# Autodesk Inventor assembly: boto suction pump
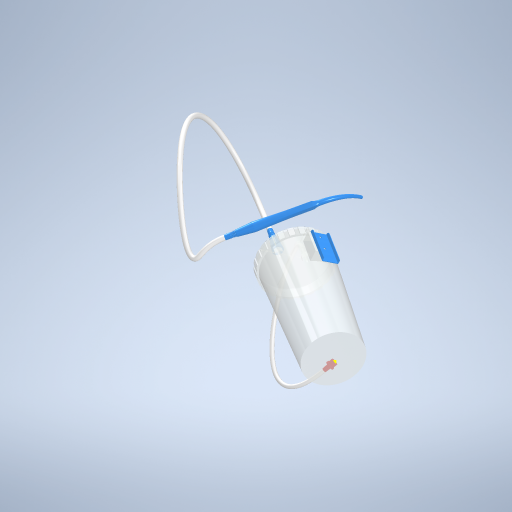
[picture p0: Inventor's stored thumbnail of the model, 512x512]
Saved by Autodesk Inventor 2024 (Build 280153000, 153)
## iProperties
Created: 2023-03-28
Part Number: boto suction pump
Description: STEP AP203
Document SubType Name: Assembly
Designer: Andani Tri
Sending System: SolidWorks 2019
Preprocessor: SwSTEP 2.0
Title: PORTABLE SUCTION R1.STEP
Revision Number: ANY
## Documents named in this file (8)
- C:\Users\ASUS\Documents\Inventor\Tugas Akhir Stechoq\Desain Botol\boto suction pump.iam
- C:\Users\ASUS\Documents\Inventor\Tugas Akhir Stechoq\Desain Botol\Tabung.ipt
- C:\Users\ASUS\Documents\Inventor\Tugas Akhir Stechoq\Desain Botol\PS 011 R1.ipt
- C:\Users\ASUS\Documents\Inventor\Tugas Akhir Stechoq\Desain Botol\NIPPLE.ipt
- C:\Users\ASUS\Documents\Inventor\Tugas Akhir Stechoq\Desain Botol\HOSE 1^PORTABLE SUCTION R1.ipt
- C:\Users\ASUS\Documents\Inventor\Tugas Akhir Stechoq\Desain Botol\NIPPLE 2.ipt
- C:\Users\ASUS\Documents\Inventor\Tugas Akhir Stechoq\Desain Botol\NIPPLE SUCTION.ipt
- C:\Users\ASUS\Documents\Inventor\Tugas Akhir Stechoq\Desain Botol\HOSE 2^PORTABLE SUCTION R1.ipt
## Components (7 placed, 7 different names)
1. Tabung_37 — Mate:5, Mate:6, Rotation:1, Mate:7, Mate:8, Mate:11, Mate:12, Mate:13, Rotation:2
2. PS 011 R1_38 — Mate:11, Mate:12, Mate:13
3. NIPPLE_52 — Mate:14, Mate:15
4. HOSE 1^PORTABLE SUCTION R1_53 — Mate:7, Mate:8, Mate:14, Mate:15, Rotation:2
5. NIPPLE 2_54 — Mate:1, Mate:2, Mate:5, Mate:6, Rotation:1
6. NIPPLE SUCTION_55 — Mate:3, Mate:4
7. HOSE 2^PORTABLE SUCTION R1_56 — Mate:1, Mate:2, Mate:3, Mate:4
## Relationships (15: Mate 13, RelateRotation 2)
- Mate:1: NIPPLE 2_54 ↔ HOSE 2^PORTABLE SUCTION R1_56
- Mate:2: NIPPLE 2_54 ↔ HOSE 2^PORTABLE SUCTION R1_56
- Mate:3: NIPPLE SUCTION_55 ↔ HOSE 2^PORTABLE SUCTION R1_56
- Mate:4: NIPPLE SUCTION_55 ↔ HOSE 2^PORTABLE SUCTION R1_56
- Mate:5: Tabung_37 ↔ NIPPLE 2_54
- Mate:6: Tabung_37 ↔ NIPPLE 2_54
- Rotation:1 [RelateRotation] (1 ul): Tabung_37 ↔ NIPPLE 2_54
- Mate:7: Tabung_37 ↔ HOSE 1^PORTABLE SUCTION R1_53
- Mate:8: Tabung_37 ↔ HOSE 1^PORTABLE SUCTION R1_53
- Mate:11: Tabung_37 ↔ PS 011 R1_38
- Mate:12: Tabung_37 ↔ PS 011 R1_38
- Mate:13: Tabung_37 ↔ PS 011 R1_38
- Mate:14: NIPPLE_52 ↔ HOSE 1^PORTABLE SUCTION R1_53
- Mate:15: NIPPLE_52 ↔ HOSE 1^PORTABLE SUCTION R1_53
- Rotation:2 [RelateRotation] (1 ul): Tabung_37 ↔ HOSE 1^PORTABLE SUCTION R1_53
